(part 1 of 2)
# Autodesk Inventor assembly: EPS
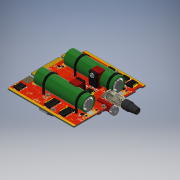
[picture p0: Inventor's stored thumbnail of the model, 180x180]
Saved by Autodesk Inventor 2018 (Build 220112000, 112)
## iProperties
Created: 2018-05-29
Part Number: EPS
Document SubType Name: Assembly
Designer: Bradley
Mass: 141.712 g
Surface Area: 416.928 cm^2
Volume: 50.0199 cm^3
Density: 2.83312 g/cm^3
Author: Bradley
## Documents named in this file (69)
- C:\Users\Bradley\Documents\GitHub\CougSat1-Hardware\CougSat1-PowerBoard\CADModel\Native\EPS.iam
- C:\Users\Bradley\Documents\GitHub\CougSat1-Hardware\CougSat1-PowerBoard\CADModel\Native\EPS_PCB.ipt
- C:\Users\Bradley\Documents\GitHub\Resources\SupplierDocuments\01 - Battery\01-0001\01-0001.ipt
- C:\Users\Bradley\Documents\GitHub\CougSat1-Hardware\CougSat1-PowerBoard\CADModel\Native\EPS_RBFPinHolder.ipt
- C:\Users\Bradley\Documents\GitHub\Resources\SupplierDocuments\25 - Resistor THT\25-10.0\25-10.0.ipt
- C:\Users\Bradley\Documents\GitHub\CougSat1-Hardware\CougSat1-PowerBoard\CADModel\Native\EPS_BatteryTab.ipt
- C:\Users\Bradley\Documents\GitHub\CougSat1-Hardware\CougSat1-PowerBoard\CADModel\Native\EPS_BatteyTie.ipt
- C:\Users\Bradley\Documents\GitHub\Resources\SupplierDocuments\04 - Connectors SMT\04-0004\04-0004.ipt
- C:\Users\Bradley\Documents\GitHub\CougSat1-Hardware\CougSat1-PowerBoard\CADModel\Native\EPS_BatteryHeatsink.ipt
- C:\Users\Bradley\Documents\GitHub\Resources\SupplierDocuments\48 - Hardware\48-0040\48-0040.ipt
- C:\Users\Bradley\Documents\GitHub\Resources\SupplierDocuments\48 - Hardware\48-0075\48-0075.ipt
- C:\Users\Bradley\Documents\GitHub\Resources\SupplierDocuments\48 - Hardware\48-0030\48-0030.ipt
- C:\Users\Bradley\Documents\GitHub\Resources\SupplierDocuments\49 - Electromechanical\49-0004\49-0004.ipt
- C:\Users\Bradley\Documents\GitHub\Resources\SupplierDocuments\04 - Connectors SMT\04-0001\04-0001.iam
- C:\Users\Bradley\Documents\GitHub\Resources\SupplierDocuments\04 - Connectors SMT\04-0007\04-0007.iam
- C:\Users\Bradley\Documents\GitHub\Resources\SupplierDocuments\05 - Connectors THT\05-0010\05-0010.iam
- C:\Users\Bradley\Documents\GitHub\Resources\SupplierDocuments\21 - Resistor 1608\21-0000\21-0000.ipt
- C:\Users\Bradley\Documents\GitHub\Resources\SupplierDocuments\21 - Resistor 1608\21-1201\21-1201.ipt
- C:\Users\Bradley\Documents\GitHub\Resources\SupplierDocuments\21 - Resistor 1608\21-1001\21-1001.ipt
- C:\Users\Bradley\Documents\GitHub\Resources\SupplierDocuments\21 - Resistor 1608\21-2201\21-2201.ipt
- C:\Users\Bradley\Documents\GitHub\Resources\SupplierDocuments\21 - Resistor 1608\21-4754\21-4754.ipt
- C:\Users\Bradley\Documents\GitHub\Resources\SupplierDocuments\21 - Resistor 1608\21-1002\21-1002.ipt
- C:\Users\Bradley\Documents\GitHub\Resources\SupplierDocuments\21 - Resistor 1608\21-1500\21-1500.ipt
- C:\Users\Bradley\Documents\GitHub\Resources\SupplierDocuments\21 - Resistor 1608\21-1583\21-1583.ipt
- C:\Users\Bradley\Documents\GitHub\Resources\SupplierDocuments\21 - Resistor 1608\21-3300\21-3300.ipt
- C:\Users\Bradley\Documents\GitHub\Resources\SupplierDocuments\21 - Resistor 1608\21-3603\21-3603.ipt
- C:\Users\Bradley\Documents\GitHub\Resources\SupplierDocuments\21 - Resistor 1608\21-4700\21-4700.ipt
- C:\Users\Bradley\Documents\GitHub\Resources\SupplierDocuments\21 - Resistor 1608\21-5363\21-5363.ipt
- C:\Users\Bradley\Documents\GitHub\Resources\SupplierDocuments\21 - Resistor 1608\21-6203\21-6203.ipt
- C:\Users\Bradley\Documents\GitHub\Resources\SupplierDocuments\21 - Resistor 1608\21-7500\21-7500.ipt
- C:\Users\Bradley\Documents\GitHub\Resources\SupplierDocuments\26 - Resistor Misc\26-0007\26-0007.ipt
- C:\Users\Bradley\Documents\GitHub\Resources\SupplierDocuments\26 - Resistor Misc\26-0000\26-0000.ipt
- C:\Users\Bradley\Documents\GitHub\Resources\SupplierDocuments\26 - Resistor Misc\26-0001\26-0001.ipt
- C:\Users\Bradley\Documents\GitHub\Resources\SupplierDocuments\26 - Resistor Misc\26-0008\26-0008.ipt
- C:\Users\Bradley\Documents\GitHub\Resources\SupplierDocuments\11 - Capacitor Ceramic 1608\11-105A\11-105A.ipt
- C:\Users\Bradley\Documents\GitHub\Resources\SupplierDocuments\16 - Capacitor Tantalum SMT\16-475A\16-475A.ipt
- C:\Users\Bradley\Documents\GitHub\Resources\SupplierDocuments\11 - Capacitor Ceramic 1608\11-4.7A\11-4.7A.ipt
- C:\Users\Bradley\Documents\GitHub\Resources\SupplierDocuments\11 - Capacitor Ceramic 1608\11-8.0A\11-8.0A.ipt
- C:\Users\Bradley\Documents\GitHub\Resources\SupplierDocuments\11 - Capacitor Ceramic 1608\11-106A\11-106A.ipt
- C:\Users\Bradley\Documents\GitHub\Resources\SupplierDocuments\11 - Capacitor Ceramic 1608\11-103A\11-103A.ipt
- C:\Users\Bradley\Documents\GitHub\Resources\SupplierDocuments\11 - Capacitor Ceramic 1608\11-150A\11-150A.ipt
- C:\Users\Bradley\Documents\GitHub\Resources\SupplierDocuments\11 - Capacitor Ceramic 1608\11-104A\11-104A.ipt
- C:\Users\Bradley\Documents\GitHub\Resources\SupplierDocuments\11 - Capacitor Ceramic 1608\11-471A\11-471A.ipt
- C:\Users\Bradley\Documents\GitHub\Resources\SupplierDocuments\34 - Inductor 3225 and larger\34-472A\34-472A.ipt
- C:\Users\Bradley\Documents\GitHub\Resources\SupplierDocuments\40 - Crystal SMT\40-805A\40-805A.ipt
- C:\Users\Bradley\Documents\GitHub\Resources\SupplierDocuments\23 - Resistor 3216\23-0.01\23-0.01.ipt
- C:\Users\Bradley\Documents\GitHub\Resources\SupplierDocuments\23 - Resistor 3216\23-12m0\23-12m0.ipt
- C:\Users\Bradley\Documents\GitHub\Resources\SupplierDocuments\40 - Crystal SMT\40-323A\40-323A.ipt
- C:\Users\Bradley\Documents\GitHub\Resources\SupplierDocuments\16 - Capacitor Tantalum SMT\16-227A\16-227A.ipt
- C:\Users\Bradley\Documents\GitHub\Resources\SupplierDocuments\27 - Conversion IC\27-0003\27-0003.ipt
- C:\Users\Bradley\Documents\GitHub\Resources\SupplierDocuments\27 - Conversion IC\27-0004\27-0004.ipt
- C:\Users\Bradley\Documents\GitHub\Resources\SupplierDocuments\08 - Amplifier (excluding RF)\08-0002\08-0002.ipt
- C:\Users\Bradley\Documents\GitHub\Resources\SupplierDocuments\60 - Power IC\60-0006\60-0006.ipt
- C:\Users\Bradley\Documents\GitHub\Resources\SupplierDocuments\56 - Transistor FET\56-0002\56-0002.ipt
- C:\Users\Bradley\Documents\GitHub\Resources\SupplierDocuments\56 - Transistor FET\56-0007\56-0007.ipt
- C:\Users\Bradley\Documents\GitHub\Resources\SupplierDocuments\56 - Transistor FET\56-0005\56-0005.ipt
- C:\Users\Bradley\Documents\GitHub\Resources\SupplierDocuments\63 - LED SMT\63-0001\63-0001.ipt
- C:\Users\Bradley\Documents\GitHub\Resources\SupplierDocuments\08 - Amplifier (excluding RF)\08-0003\08-0003.ipt
- C:\Users\Bradley\Documents\GitHub\Resources\SupplierDocuments\60 - Power IC\60-0015\60-0015.ipt
- C:\Users\Bradley\Documents\GitHub\Resources\SupplierDocuments\51 - Diode Schottky\51-0002\51-0002.ipt
- C:\Users\Bradley\Documents\GitHub\Resources\SupplierDocuments\51 - Diode Schottky\51-0001\51-0001.ipt
- C:\Users\Bradley\Documents\GitHub\Resources\SupplierDocuments\61 - µController (and CLPD, FPGA,  etc.)\61-0002\61-0002.ipt
- C:\Users\Bradley\Documents\GitHub\Resources\SupplierDocuments\60 - Power IC\60-0014\60-0014.ipt
- C:\Users\Bradley\Documents\GitHub\Resources\SupplierDocuments\60 - Power IC\60-0004\60-0004.ipt
- C:\Users\Bradley\Documents\GitHub\Resources\SupplierDocuments\09 - Communication IC\09-0001\09-0001.ipt
- C:\Users\Bradley\Documents\GitHub\Resources\SupplierDocuments\13 - Capacitor Ceramic 3216\13-106A\13-106A.ipt
- C:\Users\Bradley\Documents\GitHub\Resources\SupplierDocuments\36 - Ferrite\36-152A\36-152A.ipt
- C:\Users\Bradley\Documents\GitHub\CougSat1-Hardware\CougSat1-PowerBoard\CADModel\Native\EPS_RegulatorHeatsink-A.ipt
- C:\Users\Bradley\Documents\GitHub\CougSat1-Hardware\CougSat1-PowerBoard\CADModel\Native\EPS_RegulatorHeatsink-B.ipt
## Components (388 placed, 68 different names)
1. 36-152A:1 — Mate:1417, Mate:1418, Mate:1419
2. 13-106A:8 — Mate:1406, Mate:1416, Flush:1332
3. 13-106A:7 — Mate:1405, Mate:1414, Mate:1415
4. 13-106A:6 — Mate:1404, Mate:1413, Flush:1331
5. 13-106A:5 — Mate:1403, Mate:1412, Flush:1330
6. 13-106A:4 — Mate:1402, Mate:1411, Flush:1329
7. 13-106A:3 — Mate:1401, Mate:1409, Mate:1410
8. 13-106A:2 — Mate:1400, Mate:1408, Flush:1328
9. 13-106A:1 — Mate:1399, Mate:1407, Flush:1327
10. 09-0001:5 — Mate:1392, Flush:1325, Flush:1326
11. 09-0001:4 — Mate:1391, Flush:1323, Flush:1324
12. 09-0001:3 — Mate:1390, Flush:1321, Flush:1322
13. 09-0001:2 — Mate:1389, Mate:1397, Mate:1398
14. 09-0001:1 — Mate:1388, Mate:1395, Mate:1396
15. 60-0004:2 — Mate:1387, Flush:1320, Mate:1394
16. 60-0004:1 — Mate:1386, Flush:1319, Mate:1393
17. 60-0014:26 — Mate:1313, Flush:1318, Mate:1385
18. 60-0014:25 — Mate:1314, Flush:1317, Mate:1384
19. 60-0014:24 — Mate:1315, Mate:1382, Mate:1383
20. 60-0014:23 — Mate:1316, Flush:1316, Mate:1381
21. 60-0014:22 — Mate:1317, Flush:1315, Mate:1380
22. 60-0014:21 — Mate:1318, Mate:1378, Mate:1379
23. 60-0014:20 — Mate:1319, Mate:1376, Mate:1377
24. 60-0014:19 — Mate:1320, Mate:1374, Mate:1375
25. 60-0014:18 — Mate:1321, Mate:1372, Mate:1373
26. 60-0014:17 — Mate:1322, Mate:1370, Mate:1371
27. 60-0014:16 — Mate:1323, Mate:1368, Mate:1369
28. 60-0014:15 — Mate:1324, Mate:1366, Mate:1367
29. 60-0014:14 — Mate:1325, Mate:1364, Mate:1365
30. 60-0014:13 — Mate:1326, Mate:1362, Mate:1363
31. 60-0014:12 — Mate:1327, Mate:1360, Mate:1361
32. 60-0014:11 — Mate:1328, Mate:1358, Mate:1359
33. 60-0014:10 — Mate:1329, Mate:1356, Mate:1357
34. 60-0014:9 — Mate:1330, Mate:1354, Mate:1355
35. 60-0014:8 — Mate:1331, Mate:1352, Mate:1353
36. 60-0014:7 — Mate:1332, Mate:1350, Mate:1351
37. 60-0014:6 — Mate:1333, Mate:1348, Mate:1349
38. 60-0014:5 — Mate:1334, Mate:1346, Mate:1347
39. 60-0014:4 — Mate:1335, Mate:1344, Mate:1345
40. 60-0014:3 — Mate:1336, Mate:1342, Mate:1343
41. 60-0014:2 — Mate:1337, Mate:1340, Mate:1341
42. 60-0014:1 — Mate:1338, Flush:1314, Mate:1339
43. 61-0002:1 — Mate:1312, Flush:1312, Flush:1313
44. 51-0001:1 — Mate:1309, Mate:1310, Mate:1311
45. 51-0002:2 — Mate:1307, Mate:1308, Flush:1311
46. 51-0002:1 — Mate:1306, Flush:1309, Flush:1310
47. 60-0015:20 — Mate:1283, Mate:1305, Flush:1302
48. 60-0015:19 — Mate:1282, Mate:1303, Mate:1304
49. 60-0015:18 — Mate:1281, Mate:1301, Mate:1302
50. 60-0015:17 — Mate:1280, Mate:1300, Flush:1301
51. 60-0015:16 — Mate:1279, Mate:1299, Flush:1300
52. 60-0015:15 — Mate:1278, Flush:1299, Mate:1298
53. 60-0015:14 — Mate:1277, Flush:1298, Mate:1297
54. 60-0015:13 — Mate:1276, Flush:1297, Mate:1296
55. 60-0015:12 — Mate:1275, Flush:1296, Mate:1295
56. 60-0015:11 — Mate:1274, Mate:1294, Flush:1295
57. 60-0015:10 — Mate:1273, Mate:1293, Flush:1294
58. 60-0015:9 — Mate:1272, Mate:1292, Flush:1293
59. 60-0015:8 — Mate:1271, Mate:1291, Flush:1292
60. 60-0015:7 — Mate:1270, Flush:1291, Mate:1290
61. 60-0015:6 — Mate:1269, Flush:1290, Mate:1289
62. 60-0015:5 — Mate:1268, Flush:1289, Mate:1288
63. 60-0015:4 — Mate:1267, Flush:1288, Mate:1287
64. 60-0015:3 — Mate:1266, Mate:1286, Flush:975
65. 60-0015:2 — Mate:1265, Mate:1285, Flush:974
66. 60-0015:1 — Mate:1264, Mate:1284, Flush:973
67. 08-0003:8 — Mate:1245, Mate:1262, Mate:1263
68. 08-0003:7 — Mate:1246, Mate:1260, Mate:1261
69. 08-0003:6 — Mate:1247, Flush:972, Mate:1259
70. 08-0003:5 — Mate:1248, Flush:971, Mate:1258
71. 08-0003:4 — Mate:1249, Mate:1257, Flush:970
72. 08-0003:3 — Mate:1250, Mate:1255, Mate:1256
73. 08-0003:2 — Mate:1251, Flush:968, Flush:969
74. 08-0003:1 — Mate:1252, Mate:1253, Mate:1254
75. 63-0001:5 — Mate:1234, Mate:1243, Mate:1244
76. 63-0001:4 — Mate:1233, Mate:1241, Mate:1242
77. 63-0001:3 — Mate:1232, Mate:1239, Mate:1240
78. 63-0001:2 — Mate:1231, Mate:1237, Mate:1238
79. 63-0001:1 — Mate:1230, Mate:1235, Mate:1236
80. 56-0005:2 — Mate:1224, Mate:1227, Mate:1228
81. 56-0005:1 — Mate:1225, Mate:1226, Flush:966
82. 56-0007:2 — Mate:1221, Mate:1223, Flush:965
83. 56-0007:1 — Mate:1220, Mate:1222, Flush:964
84. 56-0002:4 — Mate:1215, Mate:1219, Flush:963
85. 56-0002:3 — Mate:1214, Mate:1218, Flush:962
86. 56-0002:2 — Mate:1213, Flush:961, Mate:1217
87. 56-0002:1 — Mate:1212, Flush:960, Mate:1216
88. 60-0006:2 — Mate:1208, Mate:1211, Flush:959
89. 60-0006:1 — Mate:1207, Mate:1209, Mate:1210
90. 08-0002:3 — Mate:1202, Mate:1205, Mate:1206
91. 08-0002:2 — Mate:1201, Flush:958, Mate:1204
92. 08-0002:1 — Mate:1200, Mate:1203, Flush:957
93. 27-0004:3 — Mate:1193, Mate:1198, Mate:1199
94. 27-0004:2 — Mate:1192, Mate:1196, Mate:1197
95. 27-0004:1 — Mate:1191, Mate:1194, Mate:1195
96. 27-0003:5 — Mate:1183, Mate:1189, Mate:1190
97. 27-0003:4 — Mate:1182, Mate:1187, Mate:1188
98. 27-0003:3 — Mate:1181, Mate:1186, Flush:956
99. 27-0003:2 — Mate:1180, Mate:1185, Flush:955
100. 27-0003:1 — Mate:1179, Flush:954, Mate:1184
101. 16-227A:3 — Mate:1174, Mate:1177, Mate:1178
102. 16-227A:2 — Mate:1173, Flush:953, Mate:1176
103. 16-227A:1 — Mate:1172, Flush:952, Mate:1175
104. 40-323A:1 — Mate:1170, Mate:1171, Flush:951
105. 23-12m0:8 — Mate:1149, Mate:1160, Mate:1161
106. 23-12m0:7 — Mate:1150, Mate:1159, Flush:950
107. 23-12m0:6 — Mate:1151, Mate:1158, Flush:949
108. 23-12m0:5 — Mate:1152, Mate:1157, Flush:948
109. 23-12m0:4 — Mate:1153, Mate:1168, Mate:1169
110. 23-12m0:3 — Mate:1154, Mate:1166, Mate:1167
111. 23-12m0:2 — Mate:1155, Mate:1164, Mate:1165
112. 23-12m0:1 — Mate:1156, Mate:1162, Mate:1163
113. 23-0.01:4 — Mate:1144, Mate:1148, Flush:947
114. 23-0.01:3 — Mate:1145, Mate:1146, Mate:1147
115. 23-0.01:2 — Mate:1139, Mate:1142, Mate:1143
116. 23-0.01:1 — Mate:1138, Mate:1140, Mate:1141
117. 40-805A:1 — Mate:1136, Mate:1137, Flush:946
118. 34-472A:2 — Mate:1131, Mate:1134, Mate:1135
119. 34-472A:1 — Mate:1130, Mate:1132, Mate:1133
120. 11-471A:2 — Mate:1126, Mate:1128, Mate:1129
121. 11-471A:1 — Mate:1125, Mate:1127, Flush:945
122. 11-104A:63 — Mate:1030, Mate:1124, Flush:944
123. 11-104A:62 — Mate:1029, Mate:1123, Flush:943
124. 11-104A:61 — Mate:1028, Mate:1122, Flush:942
125. 11-104A:60 — Mate:1027, Mate:1120, Mate:1121
126. 11-104A:59 — Mate:1026, Mate:1119, Flush:941
127. 11-104A:58 — Mate:1025, Mate:1117, Mate:1118
128. 11-104A:57 — Mate:1024, Mate:1115, Mate:1116
129. 11-104A:56 — Mate:1023, Mate:1114, Flush:940
130. 11-104A:55 — Mate:1022, Mate:1112, Mate:1113
131. 11-104A:54 — Mate:1021, Mate:1111, Flush:939
132. 11-104A:53 — Mate:1020, Mate:1110, Flush:938
133. 11-104A:52 — Mate:1019, Mate:1109, Flush:937
134. 11-104A:51 — Mate:1018, Mate:1108, Flush:936
135. 11-104A:50 — Mate:1017, Mate:1106, Mate:1107
136. 11-104A:49 — Mate:1016, Mate:1105, Flush:935
137. 11-104A:48 — Mate:1015, Mate:1104, Flush:934
138. 11-104A:47 — Mate:1014, Mate:1103, Flush:933
139. 11-104A:46 — Mate:1013, Mate:1102, Flush:932
140. 11-104A:45 — Mate:1012, Mate:1100, Mate:1101
141. 11-104A:44 — Mate:1011, Mate:1098, Mate:1099
142. 11-104A:43 — Mate:1010, Mate:1097, Flush:931
143. 11-104A:42 — Mate:1009, Mate:1095, Mate:1096
144. 11-104A:41 — Mate:1008, Mate:1093, Mate:1094
145. 11-104A:40 — Mate:1007, Mate:1091, Mate:1092
146. 11-104A:39 — Mate:1006, Mate:1090, Flush:930
147. 11-104A:38 — Mate:1005, Mate:1088, Mate:1089
148. 11-104A:37 — Mate:1004, Mate:1086, Mate:1087
149. 11-104A:36 — Mate:1003, Mate:1084, Mate:1085
150. 11-104A:35 — Mate:1002, Mate:1082, Mate:1083
151. 11-104A:34 — Mate:1001, Mate:1080, Mate:1081
152. 11-104A:33 — Mate:1000, Mate:1079, Flush:929
153. 11-104A:32 — Mate:999, Mate:1078, Flush:928
154. 11-104A:31 — Mate:998, Mate:1077, Flush:927
155. 11-104A:30 — Mate:997, Mate:1075, Mate:1076
156. 11-104A:29 — Mate:996, Mate:1073, Mate:1074
157. 11-104A:28 — Mate:995, Mate:1071, Mate:1072
158. 11-104A:27 — Mate:994, Mate:1070, Flush:926
159. 11-104A:26 — Mate:993, Mate:1069, Flush:925
160. 11-104A:25 — Mate:992, Mate:1067, Mate:1068
161. 11-104A:24 — Mate:991, Mate:1065, Mate:1066
162. 11-104A:23 — Mate:990, Mate:1064, Flush:924
163. 11-104A:22 — Mate:989, Mate:1062, Mate:1063
164. 11-104A:21 — Mate:988, Mate:1061, Flush:923
165. 11-104A:20 — Mate:987, Mate:1060, Flush:922
166. 11-104A:19 — Mate:986, Mate:1058, Mate:1059
167. 11-104A:18 — Mate:985, Mate:1057, Flush:921
168. 11-104A:17 — Mate:984, Mate:1056, Flush:920
169. 11-104A:16 — Mate:983, Mate:1055, Flush:919
170. 11-104A:15 — Mate:982, Mate:1053, Mate:1054
171. 11-104A:14 — Mate:981, Mate:1052, Flush:918
172. 11-104A:13 — Mate:980, Mate:1050, Mate:1051
173. 11-104A:12 — Mate:979, Mate:1048, Mate:1049
174. 11-104A:11 — Mate:978, Mate:1046, Mate:1047
175. 11-104A:10 — Mate:977, Mate:1044, Mate:1045
176. 11-104A:9 — Mate:976, Mate:1042, Mate:1043
177. 11-104A:8 — Mate:975, Mate:1041, Flush:917
178. 11-104A:7 — Mate:974, Mate:1039, Mate:1040
179. 11-104A:6 — Mate:973, Mate:1038, Flush:916
180. 11-104A:5 — Mate:972, Mate:1037, Flush:915
181. 11-104A:4 — Mate:971, Mate:1036, Flush:914
182. 11-104A:3 — Mate:970, Mate:1034, Mate:1035
183. 11-104A:2 — Mate:969, Mate:1032, Mate:1033
184. 11-104A:1 — Mate:968, Mate:1031, Flush:913
185. 11-150A:2 — Mate:961, Mate:966, Mate:967
186. 11-150A:1 — Mate:960, Mate:964, Mate:965
187. 11-103A:1 — Mate:959, Mate:962, Mate:963
188. 11-106A:29 — Mate:924, Mate:957, Mate:958
189. 11-106A:28 — Mate:923, Mate:956, Flush:912
190. 11-106A:27 — Mate:922, Mate:955, Flush:911
191. 11-106A:26 — Mate:921, Mate:953, Mate:954
192. 11-106A:25 — Mate:920, Mate:952, Flush:910
193. 11-106A:24 — Mate:919, Mate:950, Mate:951
194. 11-106A:23 — Mate:918, Mate:948, Mate:949
195. 11-106A:22 — Mate:917, Mate:947, Flush:909
196. 11-106A:21 — Mate:916, Mate:945, Mate:946
197. 11-106A:20 — Mate:915, Mate:944, Flush:908
198. 11-106A:19 — Mate:914, Mate:943, Flush:907
199. 11-106A:18 — Mate:913, Mate:942, Flush:906
200. 11-106A:17 — Mate:912, Mate:941, Flush:905
201. 11-106A:16 — Mate:911, Mate:940, Flush:904
202. 11-106A:15 — Mate:910, Mate:939, Flush:903
203. 11-106A:14 — Mate:909, Mate:938, Flush:902
204. 11-106A:13 — Mate:908, Mate:937, Flush:901
205. 11-106A:12 — Mate:907, Mate:936, Flush:900
206. 11-106A:11 — Mate:906, Mate:935, Flush:899
207. 11-106A:10 — Mate:905, Mate:934, Flush:898
208. 11-106A:9 — Mate:904, Mate:933, Flush:897
209. 11-106A:8 — Mate:903, Mate:932, Flush:896
210. 11-106A:7 — Mate:902, Mate:931, Flush:895
211. 11-106A:6 — Mate:901, Mate:930, Flush:894
212. 11-106A:5 — Mate:900, Mate:929, Flush:893
213. 11-106A:4 — Mate:899, Mate:928, Flush:892
214. 11-106A:3 — Mate:898, Mate:927, Flush:891
215. 11-106A:2 — Mate:897, Mate:926, Flush:890
216. 11-106A:1 — Mate:896, Mate:925, Flush:889
217. 11-8.0A:2 — Mate:889, Mate:894, Mate:895
218. 11-8.0A:1 — Mate:888, Mate:892, Mate:893
219. 11-4.7A:2 — Mate:887, Mate:891, Flush:888
220. 11-4.7A:1 — Mate:886, Mate:890, Flush:887
221. 16-475A:1 — Mate:884, Flush:886, Mate:885
222. 11-105A:26 — Mate:848, Mate:882, Mate:883
223. 11-105A:25 — Mate:847, Mate:881, Flush:103
224. 11-105A:24 — Mate:846, Mate:879, Mate:880
225. 11-105A:23 — Mate:845, Mate:878, Flush:102
226. 11-105A:22 — Mate:844, Mate:877, Flush:101
227. 11-105A:21 — Mate:843, Mate:876, Flush:100
228. 11-105A:20 — Mate:842, Mate:875, Flush:99
229. 11-105A:19 — Mate:841, Mate:874, Flush:98
230. 11-105A:18 — Mate:840, Mate:872, Mate:873
231. 11-105A:17 — Mate:839, Mate:871, Flush:97
232. 11-105A:16 — Mate:838, Mate:869, Mate:870
233. 11-105A:15 — Mate:837, Mate:867, Mate:868
234. 11-105A:14 — Mate:836, Mate:866, Flush:96
235. 11-105A:13 — Mate:835, Mate:865, Flush:95
236. 11-105A:12 — Mate:834, Mate:864, Flush:94
237. 11-105A:11 — Mate:833, Mate:863, Flush:93
238. 11-105A:10 — Mate:832, Mate:862, Flush:92
239. 11-105A:9 — Mate:831, Mate:861, Flush:91
240. 11-105A:8 — Mate:830, Mate:860, Flush:90
241. 11-105A:7 — Mate:829, Mate:859, Flush:89
242. 11-105A:6 — Mate:828, Mate:857, Mate:858
243. 11-105A:5 — Mate:827, Mate:855, Mate:856
244. 11-105A:4 — Mate:826, Mate:854, Flush:88
245. 11-105A:3 — Mate:825, Mate:853, Flush:87
246. 11-105A:2 — Mate:824, Mate:851, Mate:852
247. 11-105A:1 — Mate:823, Mate:849, Mate:850
248. 26-0008:14 — Mate:820, Mate:822, Flush:86
249. 26-0008:13 — Mate:819, Mate:821, Flush:85
250. 26-0008:12 — Mate:796, Mate:817, Mate:818
251. 26-0008:11 — Mate:795, Mate:815, Mate:816
252. 26-0008:10 — Mate:794, Mate:813, Mate:814
253. 26-0008:9 — Mate:793, Mate:811, Mate:812
254. 26-0008:8 — Mate:792, Mate:810, Flush:84
255. 26-0008:7 — Mate:791, Mate:808, Mate:809
256. 26-0008:6 — Mate:790, Mate:806, Mate:807
257. 26-0008:5 — Mate:789, Mate:804, Mate:805
258. 26-0008:4 — Mate:788, Mate:803, Flush:83
259. 26-0008:3 — Mate:787, Mate:801, Mate:802
260. 26-0008:2 — Mate:786, Mate:799, Mate:800
261. 26-0008:1 — Mate:785, Mate:797, Mate:798
262. 26-0001:2 — Mate:782, Mate:784, Flush:82
263. 26-0001:1 — Mate:781, Mate:783, Flush:81
264. 26-0000:3 — Mate:775, Mate:780, Flush:80
265. 26-0000:2 — Mate:774, Mate:778, Mate:779
266. 26-0000:1 — Mate:776, Mate:777, Flush:79
267. 26-0007:16 — Mate:746, Mate:771, Mate:772
268. 26-0007:15 — Mate:745, Mate:769, Mate:770
269. 26-0007:14 — Mate:744, Mate:767, Mate:768
270. 26-0007:13 — Mate:743, Mate:766, Flush:78
271. 26-0007:12 — Mate:742, Mate:765, Flush:77
272. 26-0007:11 — Mate:741, Mate:764, Flush:76
273. 26-0007:10 — Mate:740, Mate:763, Flush:75
274. 26-0007:9 — Mate:739, Mate:761, Mate:762
275. 26-0007:8 — Mate:738, Mate:759, Mate:760
276. 26-0007:7 — Mate:737, Mate:757, Mate:758
277. 26-0007:6 — Mate:736, Mate:755, Mate:756
278. 26-0007:5 — Mate:735, Mate:753, Mate:754
279. 26-0007:4 — Mate:734, Mate:752, Flush:74
280. 26-0007:3 — Mate:733, Mate:750, Mate:751
281. 26-0007:2 — Mate:732, Mate:748, Mate:749
282. 26-0007:1 — Mate:731, Mate:747, Flush:73
283. 21-7500:6 — Mate:717, Mate:729, Mate:730
284. 21-7500:5 — Mate:716, Mate:727, Mate:728
285. 21-7500:4 — Mate:715, Mate:726, Flush:72
286. 21-7500:3 — Mate:714, Mate:725, Flush:71
287. 21-7500:2 — Mate:713, Mate:723, Mate:724
288. 21-7500:1 — Mate:712, Mate:721, Mate:722
289. 21-6203:2 — Mate:711, Mate:720, Flush:70
290. 21-6203:1 — Mate:710, Mate:719, Flush:69
291. 21-5363:1 — Mate:709, Mate:718, Flush:68
292. 21-4700:2 — Mate:705, Mate:708, Flush:67
293. 21-4700:1 — Mate:704, Mate:706, Mate:707
294. 21-3603:2 — Mate:698, Mate:702, Mate:703
295. 21-3603:1 — Mate:697, Mate:701, Flush:66
296. 21-3300:2 — Mate:696, Mate:700, Flush:65
297. 21-3300:1 — Mate:695, Mate:699, Flush:64
298. 21-1583:1 — Mate:692, Mate:693, Mate:694
299. 21-1500:2 — Mate:688, Mate:691, Flush:63
300. 21-1500:1 — Mate:687, Mate:689, Mate:690
301. 21-1002:4 — Mate:679, Mate:685, Mate:686
302. 21-1002:3 — Mate:678, Mate:684, Flush:62
303. 21-1002:2 — Mate:677, Mate:682, Mate:683
304. 21-1002:1 — Mate:676, Mate:680, Mate:681
305. 21-4754:4 — Mate:668, Mate:674, Mate:675
306. 21-4754:3 — Mate:667, Mate:672, Mate:673
307. 21-4754:2 — Mate:666, Mate:670, Mate:671
308. 21-4754:1 — Mate:665, Mate:669, Flush:61
309. 01-0001:1 — Flush:1, Flush:4, Mate:30, Mate:32, Mate:33, Mate:39, Flush:18, Mate:41, Mate:42, Mate:544
310. 01-0001:2 — Flush:2, Flush:3, Mate:29, Mate:31, Mate:34, Mate:40, Flush:19, Mate:43, Mate:44, Mate:545
311. 04-0001:4 [sub-assembly] — Mate:18, Mate:20, Flush:32
312. 04-0001:5 [sub-assembly] — Mate:62, Mate:550, Flush:33
313. 04-0001:6 [sub-assembly] — Mate:553, Flush:35, Mate:554
314. 04-0004:1 — Mate:57, Mate:58, Flush:28
315. 04-0007:5 [sub-assembly] — Mate:14, Flush:24, Mate:548
316. 04-0007:6 [sub-assembly] — Mate:15, Flush:25, Mate:549
317. 04-0007:7 [sub-assembly] — Mate:16, Flush:40, Flush:26
318. 04-0007:8 [sub-assembly] — Mate:17, Flush:41, Flush:27
319. 05-0010:2 [sub-assembly] — Mate:53, Flush:22, Mate:55
320. 21-0000:1 — Mate:569, Mate:570, Flush:42
321. 21-0000:2 — Mate:568, Mate:571, Flush:43
322. 21-0000:3 — Mate:567, Mate:572, Flush:44
323. 21-0000:4 — Mate:566, Mate:573, Flush:45
324. 21-0000:5 — Mate:565, Mate:574, Flush:46
325. 21-0000:6 — Mate:564, Mate:575, Flush:47
326. 21-0000:7 — Mate:563, Mate:576, Flush:48
327. 21-0000:8 — Mate:562, Mate:577, Flush:49
328. 21-0000:9 — Mate:561, Mate:578, Flush:50
329. 21-0000:10 — Mate:560, Mate:579, Mate:580
330. 21-0000:11 — Mate:559, Mate:581, Mate:582
331. 21-0000:12 — Mate:558, Mate:583, Flush:51
332. 21-0000:13 — Mate:557, Mate:584, Mate:585
333. 21-0000:14 — Mate:556, Mate:586, Flush:52
334. 21-0000:15 — Mate:555, Mate:587, Mate:588
335. 21-1201:1 — Mate:589, Mate:590, Mate:591
336. 21-1001:1 — Mate:592, Mate:601, Mate:602
337. 21-1001:2 — Mate:593, Mate:603, Flush:53
338. 21-1001:3 — Mate:594, Mate:604, Mate:605
339. 21-1001:4 — Mate:595, Mate:606, Mate:607
340. 21-1001:5 — Mate:596, Mate:608, Flush:54
341. 21-1001:6 — Mate:597, Mate:609, Flush:55
342. 21-1001:7 — Mate:598, Mate:610, Flush:56
343. 21-1001:8 — Mate:599, Mate:611, Flush:57
344. 21-1001:9 — Mate:600, Mate:612, Flush:58
345. 21-2201:1 — Mate:613, Mate:631, Flush:59
346. 21-2201:2 — Mate:614, Mate:632, Mate:633
347. 21-2201:3 — Mate:615, Mate:634, Mate:635
348. 21-2201:4 — Mate:616, Mate:636, Mate:637
349. 21-2201:5 — Mate:617, Mate:638, Mate:639
350. 21-2201:6 — Mate:618, Mate:640, Mate:641
351. 21-2201:7 — Mate:619, Mate:642, Mate:643
352. 21-2201:8 — Mate:620, Mate:644, Mate:645
353. 21-2201:9 — Mate:621, Mate:646, Mate:647
354. 21-2201:10 — Mate:622, Mate:648, Mate:649
355. 21-2201:11 — Mate:623, Mate:650, Mate:651
356. 21-2201:12 — Mate:624, Mate:652, Mate:653
357. 21-2201:13 — Mate:625, Mate:654, Mate:655
358. 21-2201:14 — Mate:626, Mate:656, Mate:657
359. 21-2201:15 — Mate:627, Mate:658, Mate:659
360. 21-2201:16 — Mate:628, Mate:660, Mate:661
361. 21-2201:17 — Mate:629, Mate:662, Mate:663
362. 21-2201:18 — Mate:630, Mate:664, Flush:60
363. 25-10.0:1 — Mate:22, Mate:25, Mate:28, Flush:29, Insert:18, Insert:19
364. 25-10.0:2 — Mate:26, Mate:28, Mate:59, Insert:15, Insert:17
365. 48-0030:1 — Insert:21
366. 48-0030:2 — Insert:4
367. 48-0030:3 — Insert:23
368. 48-0030:4 — Insert:24
369. 48-0030:5 — Insert:26
370. 48-0030:6 — Insert:25
371. 48-0040:1 — Insert:17
372. 48-0040:2 — Insert:18
373. 48-0075:1 — Insert:20
374. 49-0004:1 — Mate:546, Flush:967, Mate:1229
375. EPS_RegulatorHeatsink-A:1 — Insert:27, Insert:28
376. EPS_RegulatorHeatsink-B:1 — Insert:29, Insert:30
377. EPS_BatteryHeatsink:1 — Insert:15, Mate:545
378. EPS_BatteryHeatsink:2 — Mate:544, Insert:19
379. EPS_BatteryTab:1 — Mate:32, Mate:38, Mate:39
380. EPS_BatteryTab:2 — Mate:33, Mate:36, Flush:18
381. EPS_BatteryTab:3 — Mate:31, Mate:37, Mate:40
382. EPS_BatteryTab:4 — Mate:34, Mate:35, Flush:19
383. EPS_BatteyTie:1 — Mate:41, Mate:47, Mate:49
384. EPS_BatteyTie:2 — Mate:42, Mate:48, Mate:50
385. EPS_BatteyTie:3 — Mate:43, Mate:45, Mate:51
386. EPS_BatteyTie:4 — Mate:44, Mate:46, Mate:52
387. EPS_PCB:1 — Flush:1, Flush:2, Mate:14, Mate:15, Mate:16, Mate:17, Mate:18, Insert:4, Insert:9, Mate:22, Flush:40, Flush:41, Mate:25, Mate:26, Mate:35, Mate:36, Mate:37, Mate:38, Mate:45, Mate:46, Mate:47, Mate:48, Mate:49, Mate:50, Mate:51, Mate:52, Mate:55, Mate:57, Flush:28, Mate:62, Insert:21, Mate:546, Insert:22, Insert:23, Insert:24, Insert:25, Insert:26, Mate:553, Mate:555, Mate:556, Mate:557, Mate:558, Mate:559, Mate:560, Mate:561, Mate:562, Mate:563, Mate:564, Mate:565, Mate:566, Mate:567, Mate:568, Mate:569, Mate:589, Mate:592, Mate:593, Mate:594, Mate:595, Mate:596, Mate:597, Mate:598, Mate:599, Mate:600, Mate:613, Mate:614, Mate:615, Mate:616, Mate:617, Mate:618, Mate:619, Mate:620, Mate:621, Mate:622, Mate:623, Mate:624, Mate:625, Mate:626, Mate:627, Mate:628, Mate:629, Mate:630, Mate:665, Mate:666, Mate:667, Mate:668, Mate:676, Mate:677, Mate:678, Mate:679, Mate:687, Mate:688, Mate:692, Mate:695, Mate:696, Mate:697, Mate:698, Mate:704, Mate:705, Mate:709, Mate:710, Mate:711, Mate:712, Mate:713, Mate:714, Mate:715, Mate:716, Mate:717, Mate:731, Mate:732, Mate:733, Mate:734, Mate:735, Mate:736, Mate:737, Mate:738, Mate:739, Mate:740, Mate:741, Mate:742, Mate:743, Mate:744, Mate:745, Mate:746, Mate:774, Mate:775, Mate:776, Mate:781, Mate:782, Mate:785, Mate:786, Mate:787, Mate:788, Mate:789, Mate:790, Mate:791, Mate:792, Mate:793, Mate:794, Mate:795, Mate:796, Mate:819, Mate:820, Mate:823, Mate:824, Mate:825, Mate:826, Mate:827, Mate:828, Mate:829, Mate:830, Mate:831, Mate:832, Mate:833, Mate:834, Mate:835, Mate:836, Mate:837, Mate:838, Mate:839, Mate:840, Mate:841, Mate:842, Mate:843, Mate:844, Mate:845, Mate:846, Mate:847, Mate:848, Mate:884, Mate:886, Mate:887, Mate:888, Mate:889, Mate:896, Mate:897, Mate:898, Mate:899, Mate:900, Mate:901, Mate:902, Mate:903, Mate:904, Mate:905, Mate:906, Mate:907, Mate:908, Mate:909, Mate:910, Mate:911, Mate:912, Mate:913, Mate:914, Mate:915, Mate:916, Mate:917, Mate:918, Mate:919, Mate:920, Mate:921, Mate:922, Mate:923, Mate:924, Mate:959, Mate:960, Mate:961, Mate:968, Mate:969, Mate:970, Mate:971, Mate:972, Mate:973, Mate:974, Mate:975, Mate:976, Mate:977, Mate:978, Mate:979, Mate:980, Mate:981, Mate:982, Mate:983, Mate:984, Mate:985, Mate:986, Mate:987, Mate:988, Mate:989, Mate:990, Mate:991, Mate:992, Mate:993, Mate:994, Mate:995, Mate:996, Mate:997, Mate:998, Mate:999, Mate:1000, Mate:1001, Mate:1002, Mate:1003, Mate:1004, Mate:1005, Mate:1006, Mate:1007, Mate:1008, Mate:1009, Mate:1010, Mate:1011, Mate:1012, Mate:1013, Mate:1014, Mate:1015, Mate:1016, Mate:1017, Mate:1018, Mate:1019, Mate:1020, Mate:1021, Mate:1022, Mate:1023, Mate:1024, Mate:1025, Mate:1026, Mate:1027, Mate:1028, Mate:1029, Mate:1030, Mate:1125, Mate:1126, Mate:1130, Mate:1131, Mate:1136, Mate:1138, Mate:1139, Mate:1144, Mate:1145, Mate:1149, Mate:1150, Mate:1151, Mate:1152, Mate:1153, Mate:1154, Mate:1155, Mate:1156, Mate:1170, Mate:1172, Mate:1173, Mate:1174, Mate:1179, Mate:1180, Mate:1181, Mate:1182, Mate:1183, Mate:1191, Mate:1192, Mate:1193, Mate:1200, Mate:1201, Mate:1202, Mate:1207, Mate:1208, Mate:1212, Mate:1213, Mate:1214, Mate:1215, Mate:1220, Mate:1221, Mate:1224, Mate:1225, Mate:1230, Mate:1231, Mate:1232, Mate:1233, Mate:1234, Mate:1245, Mate:1246, Mate:1247, Mate:1248, Mate:1249, Mate:1250, Mate:1251, Mate:1252, Mate:1264, Mate:1265, Mate:1266, Mate:1267, Mate:1268, Mate:1269, Mate:1270, Mate:1271, Mate:1272, Mate:1273, Mate:1274, Mate:1275, Mate:1276, Mate:1277, Mate:1278, Mate:1279, Mate:1280, Mate:1281, Mate:1282, Mate:1283, Mate:1306, Mate:1307, Mate:1309, Mate:1312, Mate:1313, Mate:1314, Mate:1315, Mate:1316, Mate:1317, Mate:1318, Mate:1319, Mate:1320, Mate:1321, Mate:1322, Mate:1323, Mate:1324, Mate:1325, Mate:1326, Mate:1327, Mate:1328, Mate:1329, Mate:1330, Mate:1331, Mate:1332, Mate:1333, Mate:1334, Mate:1335, Mate:1336, Mate:1337, Mate:1338, Mate:1386, Mate:1387, Mate:1388, Mate:1389, Mate:1390, Mate:1391, Mate:1392, Mate:1399, Mate:1400, Mate:1401, Mate:1402, Mate:1403, Mate:1404, Mate:1405, Mate:1406, Mate:1417, Insert:27, Insert:28, Insert:29, Insert:30
388. EPS_RBFPinHolder:1 — Insert:9, Insert:20, Insert:22
## Relationships (1138: Mate 912, Flush 209, Insert 17)
- Flush:1 (-9.15 mm): 01-0001:1 ↔ EPS_PCB:1
- Flush:2 (-9.15 mm): 01-0001:2 ↔ EPS_PCB:1
- Flush:3 (-51 mm): 01-0001:2
- Flush:4 (-49 mm): 01-0001:1
- Mate:14: 04-0007:5 ↔ EPS_PCB:1
- Mate:15: 04-0007:6 ↔ EPS_PCB:1
- Mate:16: 04-0007:7 ↔ EPS_PCB:1
- Mate:17: 04-0007:8 ↔ EPS_PCB:1
- Mate:18: 04-0001:4 ↔ EPS_PCB:1
- Insert:4: 48-0030:2 ↔ EPS_PCB:1
- Insert:9: EPS_PCB:1 ↔ EPS_RBFPinHolder:1
- Mate:20 (0.3 mm): 04-0001:4
- Mate:22: 25-10.0:1 ↔ EPS_PCB:1
- Flush:40 (-54 mm): 04-0007:7 ↔ EPS_PCB:1
- Flush:41 (-73.5 mm): 04-0007:8 ↔ EPS_PCB:1
- Mate:25 (-60 mm): 25-10.0:1 ↔ EPS_PCB:1
- Mate:26: 25-10.0:2 ↔ EPS_PCB:1
- Mate:28: 25-10.0:1 ↔ 25-10.0:2
- Mate:29 (-21 mm): 01-0001:2
- Mate:30 (21 mm): 01-0001:1
- Mate:31: 01-0001:2 ↔ EPS_BatteryTab:3
- Mate:32: 01-0001:1 ↔ EPS_BatteryTab:1
- Mate:33: 01-0001:1 ↔ EPS_BatteryTab:2
- Mate:34: 01-0001:2 ↔ EPS_BatteryTab:4
- Mate:35: EPS_BatteryTab:4 ↔ EPS_PCB:1
- Mate:36: EPS_BatteryTab:2 ↔ EPS_PCB:1
- Mate:37: EPS_BatteryTab:3 ↔ EPS_PCB:1
- Mate:38: EPS_BatteryTab:1 ↔ EPS_PCB:1
- Mate:39: 01-0001:1 ↔ EPS_BatteryTab:1
- Flush:18: 01-0001:1 ↔ EPS_BatteryTab:2
- Mate:40: 01-0001:2 ↔ EPS_BatteryTab:3
- Flush:19: 01-0001:2 ↔ EPS_BatteryTab:4
- Mate:41: 01-0001:1 ↔ EPS_BatteyTie:1
- Mate:42: 01-0001:1 ↔ EPS_BatteyTie:2
- Mate:43: 01-0001:2 ↔ EPS_BatteyTie:3
- Mate:44: 01-0001:2 ↔ EPS_BatteyTie:4
- Mate:45: EPS_BatteyTie:3 ↔ EPS_PCB:1
- Mate:46: EPS_BatteyTie:4 ↔ EPS_PCB:1
- Mate:47: EPS_BatteyTie:1 ↔ EPS_PCB:1
- Mate:48: EPS_BatteyTie:2 ↔ EPS_PCB:1
- Mate:49: EPS_BatteyTie:1 ↔ EPS_PCB:1
- Mate:50: EPS_BatteyTie:2 ↔ EPS_PCB:1
- Mate:51: EPS_BatteyTie:3 ↔ EPS_PCB:1
- Mate:52: EPS_BatteyTie:4 ↔ EPS_PCB:1
- Mate:53 (13 mm): 05-0010:2
- Flush:22: 05-0010:2
- Mate:55 (1.7 mm): 05-0010:2 ↔ EPS_PCB:1
- Flush:24 (-36.75 mm): 04-0007:5
- Flush:25 (-36.75 mm): 04-0007:6
- Flush:26 (36.75 mm): 04-0007:7
- Flush:27 (36.75 mm): 04-0007:8
- Mate:57: 04-0004:1 ↔ EPS_PCB:1
- Mate:58 (6.35 mm): 04-0004:1
- Flush:28 (47 mm): 04-0004:1 ↔ EPS_PCB:1
- Mate:59 (-9.8 mm): 25-10.0:2
- Flush:29 (-9.8 mm): 25-10.0:1
- Mate:62: 04-0001:5 ↔ EPS_PCB:1
- Insert:15: 25-10.0:2 ↔ EPS_BatteryHeatsink:1
- Mate:544: 01-0001:1 ↔ EPS_BatteryHeatsink:2
- Mate:545: 01-0001:2 ↔ EPS_BatteryHeatsink:1
- Insert:17: 25-10.0:2 ↔ 48-0040:1
- Insert:18: 25-10.0:1 ↔ 48-0040:2
- Insert:19: 25-10.0:1 ↔ EPS_BatteryHeatsink:2
- Insert:20: 48-0075:1 ↔ EPS_RBFPinHolder:1
- Insert:21: 48-0030:1 ↔ EPS_PCB:1
- Mate:546: 49-0004:1 ↔ EPS_PCB:1
- Insert:22: EPS_PCB:1 ↔ EPS_RBFPinHolder:1
- Flush:32 (-58 mm): 04-0001:4
- Mate:548 (54 mm): 04-0007:5
- Mate:549 (73.5 mm): 04-0007:6
- Insert:23: 48-0030:3 ↔ EPS_PCB:1
- Insert:24: 48-0030:4 ↔ EPS_PCB:1
- Insert:25: 48-0030:6 ↔ EPS_PCB:1
- Insert:26: 48-0030:5 ↔ EPS_PCB:1
- Mate:550 (39 mm): 04-0001:5
- Flush:33 (-77 mm): 04-0001:5
- Mate:553: 04-0001:6 ↔ EPS_PCB:1
- Flush:35 (39 mm): 04-0001:6
- Mate:554 (13 mm): 04-0001:6
- Mate:555: 21-0000:15 ↔ EPS_PCB:1
- Mate:556: 21-0000:14 ↔ EPS_PCB:1
- Mate:557: 21-0000:13 ↔ EPS_PCB:1
- Mate:558: 21-0000:12 ↔ EPS_PCB:1
- Mate:559: 21-0000:11 ↔ EPS_PCB:1
- Mate:560: 21-0000:10 ↔ EPS_PCB:1
- Mate:561: 21-0000:9 ↔ EPS_PCB:1
- Mate:562: 21-0000:8 ↔ EPS_PCB:1
- Mate:563: 21-0000:7 ↔ EPS_PCB:1
- Mate:564: 21-0000:6 ↔ EPS_PCB:1
- Mate:565: 21-0000:5 ↔ EPS_PCB:1
- Mate:566: 21-0000:4 ↔ EPS_PCB:1
- Mate:567: 21-0000:3 ↔ EPS_PCB:1
- Mate:568: 21-0000:2 ↔ EPS_PCB:1
- Mate:569: 21-0000:1 ↔ EPS_PCB:1
- Mate:570 (61.2 mm): 21-0000:1
- Flush:42 (-44 mm): 21-0000:1
- Mate:571 (56.5 mm): 21-0000:2
- Flush:43 (34.4 mm): 21-0000:2
- Mate:572 (61.2 mm): 21-0000:3
- Flush:44 (44 mm): 21-0000:3
- Mate:573 (36.6 mm): 21-0000:4
- Flush:45 (-26.3 mm): 21-0000:4
- Mate:574 (54.1 mm): 21-0000:5
- Flush:46 (-37.6 mm): 21-0000:5
- Mate:575 (52.7 mm): 21-0000:6
- Flush:47 (-41 mm): 21-0000:6
- Mate:576 (54.8 mm): 21-0000:7
- Flush:48 (-6.6 mm): 21-0000:7
- Mate:577 (23.2 mm): 21-0000:8
- Flush:49 (2.4 mm): 21-0000:8
- Mate:578 (83.5 mm): 21-0000:9
- Flush:50 (4.9 mm): 21-0000:9
- Mate:579 (6 mm): 21-0000:10
- Mate:580 (45 mm): 21-0000:10
- Mate:581 (8.4 mm): 21-0000:11
- Mate:582 (79.2 mm): 21-0000:11
- Mate:583 (55.7 mm): 21-0000:12
- Flush:51 (25.2 mm): 21-0000:12
- Mate:584 (30.2 mm): 21-0000:13
- Mate:585 (50.6 mm): 21-0000:13
- Mate:586 (55.7 mm): 21-0000:14
- Flush:52 (28.6 mm): 21-0000:14
- Mate:587 (-25.7 mm): 21-0000:15
- Mate:588 (34.9 mm): 21-0000:15
- Mate:589: 21-1201:1 ↔ EPS_PCB:1
- Mate:590 (30.7 mm): 21-1201:1
- Mate:591 (19 mm): 21-1201:1
- Mate:592: 21-1001:1 ↔ EPS_PCB:1
- Mate:593: 21-1001:2 ↔ EPS_PCB:1
- Mate:594: 21-1001:3 ↔ EPS_PCB:1
- Mate:595: 21-1001:4 ↔ EPS_PCB:1
- Mate:596: 21-1001:5 ↔ EPS_PCB:1
- Mate:597: 21-1001:6 ↔ EPS_PCB:1
- Mate:598: 21-1001:7 ↔ EPS_PCB:1
- Mate:599: 21-1001:8 ↔ EPS_PCB:1
- Mate:600: 21-1001:9 ↔ EPS_PCB:1
- Mate:601 (16.7 mm): 21-1001:1
- Mate:602 (28.8 mm): 21-1001:1
- Mate:603 (82.6 mm): 21-1001:2
- Flush:53 (8.3 mm): 21-1001:2
- Mate:604 (8.4 mm): 21-1001:3
- Mate:605 (89.5 mm): 21-1001:3
- Mate:606 (6 mm): 21-1001:4
- Mate:607 (49.6 mm): 21-1001:4
- Mate:608 (81.4 mm): 21-1001:5
- Flush:54 (31.7 mm): 21-1001:5
- Mate:609 (31.6 mm): 21-1001:6
- Flush:55 (-39.4 mm): 21-1001:6
- Mate:610 (82.5 mm): 21-1001:7
- Flush:56 (-31.3 mm): 21-1001:7
- Mate:611 (44.1 mm): 21-1001:8
- Flush:57 (-8.6 mm): 21-1001:8
- Mate:612 (38.6 mm): 21-1001:9
- Flush:58 (33.6 mm): 21-1001:9
- Mate:613: 21-2201:1 ↔ EPS_PCB:1
- Mate:614: 21-2201:2 ↔ EPS_PCB:1
- Mate:615: 21-2201:3 ↔ EPS_PCB:1
- Mate:616: 21-2201:4 ↔ EPS_PCB:1
- Mate:617: 21-2201:5 ↔ EPS_PCB:1
- Mate:618: 21-2201:6 ↔ EPS_PCB:1
- Mate:619: 21-2201:7 ↔ EPS_PCB:1
- Mate:620: 21-2201:8 ↔ EPS_PCB:1
- Mate:621: 21-2201:9 ↔ EPS_PCB:1
- Mate:622: 21-2201:10 ↔ EPS_PCB:1
- Mate:623: 21-2201:11 ↔ EPS_PCB:1
- Mate:624: 21-2201:12 ↔ EPS_PCB:1
- Mate:625: 21-2201:13 ↔ EPS_PCB:1
- Mate:626: 21-2201:14 ↔ EPS_PCB:1
- Mate:627: 21-2201:15 ↔ EPS_PCB:1
- Mate:628: 21-2201:16 ↔ EPS_PCB:1
- Mate:629: 21-2201:17 ↔ EPS_PCB:1
- Mate:630: 21-2201:18 ↔ EPS_PCB:1
- Mate:631 (40.8 mm): 21-2201:1
- Flush:59 (16.9 mm): 21-2201:1
- Mate:632 (42.7 mm): 21-2201:2
- Mate:633 (19 mm): 21-2201:2
- Mate:634 (40.2 mm): 21-2201:3
- Mate:635 (26.8 mm): 21-2201:3
- Mate:636 (38.7 mm): 21-2201:4
- Mate:637 (19 mm): 21-2201:4
- Mate:638 (36.7 mm): 21-2201:5
- Mate:639 (26.8 mm): 21-2201:5
- Mate:640 (34.7 mm): 21-2201:6
- Mate:641 (19 mm): 21-2201:6
- Mate:642 (32.7 mm): 21-2201:7
- Mate:643 (26.8 mm): 21-2201:7
- Mate:644 (14.7 mm): 21-2201:8
- Mate:645 (21 mm): 21-2201:8
- Mate:646 (5.6 mm): 21-2201:9
- Mate:647 (8.5 mm): 21-2201:9
- Mate:648 (12.1 mm): 21-2201:10
- Mate:649 (28.8 mm): 21-2201:10
- Mate:650 (10.7 mm): 21-2201:11
- Mate:651 (21 mm): 21-2201:11
- Mate:652 (8.7 mm): 21-2201:12
- Mate:653 (28.8 mm): 21-2201:12
- Mate:654 (-9.4 mm): 21-2201:13
- Mate:655 (14.5 mm): 21-2201:13
- Mate:656 (28.7 mm): 21-2201:14
- Mate:657 (28.8 mm): 21-2201:14
- Mate:658 (24.7 mm): 21-2201:15
- Mate:659 (28.8 mm): 21-2201:15
- Mate:660 (22.7 mm): 21-2201:16
- Mate:661 (21 mm): 21-2201:16
- Mate:662 (18.8 mm): 21-2201:17
- Mate:663 (21 mm): 21-2201:17
- Mate:664 (86.3 mm): 21-2201:18
- Flush:60 (39.8 mm): 21-2201:18
- Mate:665: 21-4754:1 ↔ EPS_PCB:1
- Mate:666: 21-4754:2 ↔ EPS_PCB:1
- Mate:667: 21-4754:3 ↔ EPS_PCB:1
- Mate:668: 21-4754:4 ↔ EPS_PCB:1
- Mate:669 (10.2 mm): 21-4754:1
- Flush:61 (-7.9 mm): 21-4754:1
- Mate:670 (-9.6 mm): 21-4754:2
- Mate:671 (16.2 mm): 21-4754:2
- Mate:672 (5.4 mm): 21-4754:3